# Autodesk Inventor assembly: Wrist
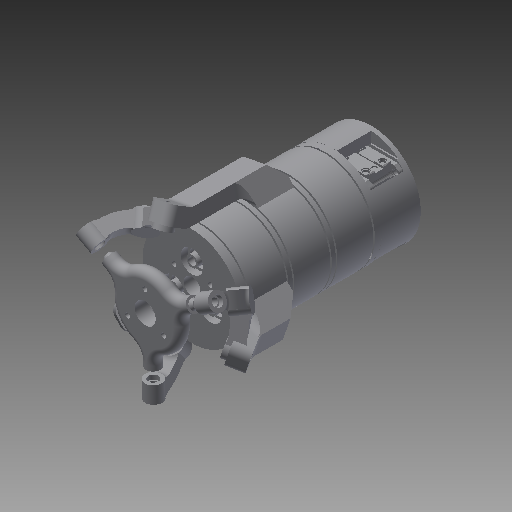
[picture p0: Inventor's stored thumbnail of the model, 512x512]
Saved by Autodesk Inventor 2019 (Build 230136000, 136)
## iProperties
Created: 2022-09-05
Part Number: Wrist
Document SubType Name: Assembly
Designer: zreik
Author: zreik
## Documents named in this file (15)
- D:\Documents\HIAST\4th year\4th Year Project\Design\Final\Inventor\Wrist.iam
- D:\Documents\HIAST\4th year\4th Year Project\Design\Final\Inventor\Base.ipt
- D:\Documents\HIAST\4th year\4th Year Project\Design\Final\Inventor\XL-320.ipt
- D:\Documents\HIAST\4th year\4th Year Project\Design\Final\Inventor\Layer1Base.ipt
- D:\Documents\HIAST\4th year\4th Year Project\Design\Final\Inventor\Layer1Gear.ipt
- D:\Documents\HIAST\4th year\4th Year Project\Design\Final\Inventor\Layer2Base.ipt
- D:\Documents\HIAST\4th year\4th Year Project\Design\Final\Inventor\Layer2Gear.ipt
- D:\Documents\HIAST\4th year\4th Year Project\Design\Final\Inventor\Layer3Base.ipt
- D:\Documents\HIAST\4th year\4th Year Project\Design\Final\Inventor\Layer3Gear.ipt
- D:\Documents\HIAST\4th year\4th Year Project\Design\Final\Inventor\Motor1Gear.ipt
- D:\Documents\HIAST\4th year\4th Year Project\Design\Final\Inventor\Motor2Gear.ipt
- D:\Documents\HIAST\4th year\4th Year Project\Design\Final\Inventor\Motor3Gear.ipt
- D:\Documents\HIAST\4th year\4th Year Project\Design\Final\Inventor\Cover.ipt
- D:\Documents\HIAST\4th year\4th Year Project\Design\Final\Inventor\Link.ipt
- D:\Documents\HIAST\4th year\4th Year Project\Design\Final\Inventor\Platform.ipt
## Components (18 placed, 14 different names)
1. Base:1 — Flush:1, Flush:2, Mate:1, Mate:2, Mate:3, Mate:4, Mate:5, Mate:6, Mate:7, Mate:8
2. Layer1Base:1 — Mate:5, Mate:6, Mate:7, Mate:9, Mate:10, Mate:16, Mate:20, Mate:22, Mate:24
3. Layer1Gear:1 — Mate:8, Mate:9, Mate:11, Mate:12, Mate:31
4. Layer2Base:1 — Mate:10, Mate:11, Mate:13, Mate:14, Mate:16, Mate:17
5. Layer2Gear:1 — Mate:12, Mate:13, Mate:15, Mate:18, Mate:30
6. Layer3Base:1 — Mate:14, Mate:15, Mate:17, Mate:19, Mate:27
7. Layer3Gear:1 — Mate:18, Mate:19, Mate:26, Mate:28, Mate:29
8. Motor1Gear:1 — Mate:20, Mate:21
9. Motor2Gear:1 — Mate:22, Mate:23
10. Motor3Gear:1 — Mate:24, Mate:25
11. Cover:1 — Mate:26, Mate:27, Mate:28, Angle:1
12. Link:1 — Mate:31, Mate:35
13. Link:2 — Mate:30, Mate:34
14. Link:3 — Mate:29, Mate:32
15. Platform:1 — Angle:1, Mate:32, Mate:34, Mate:35
16. XL-320:1 — Mate:2, Mate:3, Mate:4, Mate:23
17. XL-320:2 — Mate:21
18. XL-320:3 — Mate:25
## Component patterns: (3 elements, first: XL-320:1)
## Relationships (37: Mate 34, Flush 2, Angle 1)
- Flush:1: Base:1
- Flush:2: Base:1
- Mate:1: Base:1
- Mate:2: Base:1 ↔ XL-320:1
- Mate:3: Base:1 ↔ XL-320:1
- Mate:4: Base:1 ↔ XL-320:1
- Mate:5: Base:1 ↔ Layer1Base:1
- Mate:6: Base:1 ↔ Layer1Base:1
- Mate:7: Base:1 ↔ Layer1Base:1
- Mate:8: Base:1 ↔ Layer1Gear:1
- Mate:9: Layer1Base:1 ↔ Layer1Gear:1
- Mate:10: Layer1Base:1 ↔ Layer2Base:1
- Mate:11: Layer1Gear:1 ↔ Layer2Base:1
- Mate:12: Layer1Gear:1 ↔ Layer2Gear:1
- Mate:13: Layer2Base:1 ↔ Layer2Gear:1
- Mate:14: Layer2Base:1 ↔ Layer3Base:1
- Mate:15: Layer2Gear:1 ↔ Layer3Base:1
- Mate:16: Layer1Base:1 ↔ Layer2Base:1
- Mate:17: Layer2Base:1 ↔ Layer3Base:1
- Mate:18: Layer2Gear:1 ↔ Layer3Gear:1
- Mate:19: Layer3Base:1 ↔ Layer3Gear:1
- Mate:20: Layer1Base:1 ↔ Motor1Gear:1
- Mate:21: Motor1Gear:1 ↔ XL-320:2
- Mate:22: Layer1Base:1 ↔ Motor2Gear:1
- Mate:23: Motor2Gear:1 ↔ XL-320:1
- Mate:24: Layer1Base:1 ↔ Motor3Gear:1
- Mate:25: Motor3Gear:1 ↔ XL-320:3
- Mate:26: Layer3Gear:1 ↔ Cover:1
- Mate:27: Layer3Base:1 ↔ Cover:1
- Mate:28: Layer3Gear:1 ↔ Cover:1
- Mate:29: Layer3Gear:1 ↔ Link:3
- Mate:30: Layer2Gear:1 ↔ Link:2
- Mate:31: Layer1Gear:1 ↔ Link:1
- Angle:1 (0 deg): Cover:1 ↔ Platform:1
- Mate:32: Link:3 ↔ Platform:1
- Mate:34: Link:2 ↔ Platform:1
- Mate:35: Link:1 ↔ Platform:1
